# Autodesk Inventor assembly: Grabber and joint subassembly (1)
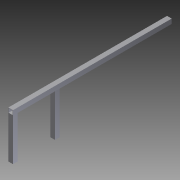
[picture p0: Inventor's stored thumbnail of the model, 180x180]
Saved by Autodesk Inventor 2011 SP1 (Build 150282100, 282)
## iProperties
Created: 2011-01-11
Part Number: Grabber and joint subassembly (1)
Document SubType Name: Assembly
Designer: 13351773
Author: 13351773
## Documents named in this file (3)
- C:\Users\Christopher\Documents\Christopher\FIRST\Inventor files\2011\linlifterarm\Grabber and joint subassembly (1).iam
- C:\Users\Christopher\Downloads\AB1-16-34-001.ipt
- C:\Users\Christopher\Downloads\AB1-16-9-001.ipt
## Components (3 placed, 2 different names)
1. AB1-16-34-001:1 — Mate:1, Flush:1, Flush:2, Mate:2, Flush:3, Flush:4
2. AB1-16-9-001:1 — Mate:2, Flush:3, Flush:4
3. AB1-16-9-001:2 — Mate:1, Flush:1, Flush:2
## Relationships (6: Flush 4, Mate 2)
- Mate:1: AB1-16-34-001:1 ↔ AB1-16-9-001:2
- Flush:1: AB1-16-34-001:1 ↔ AB1-16-9-001:2
- Flush:2: AB1-16-34-001:1 ↔ AB1-16-9-001:2
- Mate:2: AB1-16-34-001:1 ↔ AB1-16-9-001:1
- Flush:3: AB1-16-34-001:1 ↔ AB1-16-9-001:1
- Flush:4 (228.6 mm): AB1-16-34-001:1 ↔ AB1-16-9-001:1
